# Autodesk Inventor assembly: inner_miirrored
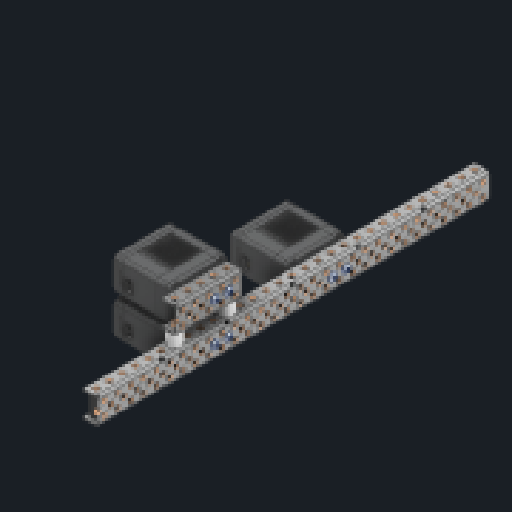
[picture p0: Inventor's stored thumbnail of the model, 512x512]
Saved by Autodesk Inventor 2025 (Build 290162000, 162)
## iProperties
Created: 2024-10-03
Part Number: inner_miirrored
Document SubType Name: Assembly
Designer: Averey Ku
Author: Averey Ku
## Documents named in this file (10)
- D:\vex_robotics_high_stakes\hardware\cad\bots\high_stakes_v2\chassis\drivebay_mirrored\inner_miirrored.iam
- D:\vex_robotics_high_stakes\hardware\cad\bots\high_stakes_v2\chassis\drivebay_mirrored\Alu C 1x2x1x30_miirrored.ipt
- D:\vex_robotics_high_stakes\hardware\cad\robpros_cad_lib\Motion\Spacers\Spacer Nylon .500 OD\NSpacer White .500 OD x .500.ipt
- D:\vex_robotics_high_stakes\hardware\cad\robpros_cad_lib\Motion\Spacers\Spacer Nylon .500 OD.ipt
- D:\vex_robotics_high_stakes\hardware\cad\bots\high_stakes_v2\chassis\drivebay_mirrored\Alu C 1x2x1x5_miirrored.ipt
- D:\vex_robotics_high_stakes\hardware\cad\bots\high_stakes_v2\chassis\drivebay_mirrored\SteelM-StarS_miirrored.iam
- D:\vex_robotics_high_stakes\hardware\cad\VEX-CAD-Inventor\Structure\Standoff\Standoff .875.ipt
- D:\vex_robotics_high_stakes\hardware\cad\VEX-CAD-Inventor\Structure\Standoff.ipt
- D:\vex_robotics_high_stakes\hardware\cad\robpros_cad_lib\Motion\Spacers\Spacer Nylon .375 OD\NSpacer .375 OD x .875.ipt
- D:\vex_robotics_high_stakes\hardware\cad\robpros_cad_lib\Motion\Spacers\Spacer Nylon .375 OD.ipt
## Components (10 placed, 6 different names)
1. Alu C 1x2x1x30_miirrored:1 — Mate:2, Insert:2, Insert:1, Mate:4, Insert:6, Insert:5, Insert:7, Insert:8, Insert:9
2. NSpacer White .500 OD x .500:1 — Insert:2, Insert:3
3. NSpacer White .500 OD x .500:2 — Insert:1, Mate:5
4. Alu C 1x2x1x5_miirrored:1 — Insert:3, Mate:3, Insert:4, Mate:5
5. SteelM-StarS_miirrored:1 [sub-assembly] — Mate:3, Insert:4
6. SteelM-StarS_miirrored:2 [sub-assembly] — Mate:4, Insert:6
7. SteelM-StarS_miirrored:3 [sub-assembly] — Insert:5
8. Standoff .875:1 — Insert:7
9. Standoff .875:2 — Insert:8
10. NSpacer .375 OD x .875:1 — Insert:9
## Relationships (13: Insert 9, Mate 4)
- Mate:2: Alu C 1x2x1x30_miirrored:1
- Insert:2: Alu C 1x2x1x30_miirrored:1 ↔ NSpacer White .500 OD x .500:1
- Insert:1: Alu C 1x2x1x30_miirrored:1 ↔ NSpacer White .500 OD x .500:2
- Insert:3: NSpacer White .500 OD x .500:1 ↔ Alu C 1x2x1x5_miirrored:1
- Mate:3: Alu C 1x2x1x5_miirrored:1 ↔ SteelM-StarS_miirrored:1
- Insert:4: Alu C 1x2x1x5_miirrored:1 ↔ SteelM-StarS_miirrored:1
- Mate:4: Alu C 1x2x1x30_miirrored:1 ↔ SteelM-StarS_miirrored:2
- Insert:6: Alu C 1x2x1x30_miirrored:1 ↔ SteelM-StarS_miirrored:2
- Insert:5: Alu C 1x2x1x30_miirrored:1 ↔ SteelM-StarS_miirrored:3
- Insert:7: Alu C 1x2x1x30_miirrored:1 ↔ Standoff .875:1
- Insert:8: Alu C 1x2x1x30_miirrored:1 ↔ Standoff .875:2
- Insert:9: Alu C 1x2x1x30_miirrored:1 ↔ NSpacer .375 OD x .875:1
- Mate:5: NSpacer White .500 OD x .500:2 ↔ Alu C 1x2x1x5_miirrored:1
